# Autodesk Inventor assembly: основа
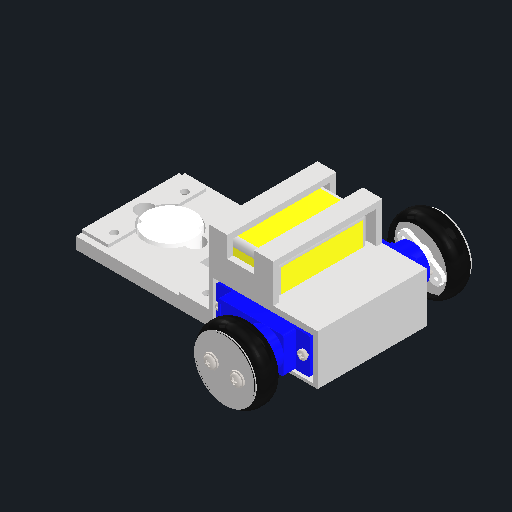
[picture p0: Inventor's stored thumbnail of the model, 512x512]
Saved by Autodesk Inventor 2022 (Build 260153000, 153)
## iProperties
Created: 2025-02-02
Part Number: основа
Document SubType Name: Assembly
Designer: Admin
Author: Admin
## Documents named in this file (7)
- D:\машина\основа.iam
- D:\abuyz lkz vfibyrb\аккум.ipt
- D:\машина\сервоприводы.iam
- D:\abuyz lkz vfibyrb\сфер.подшип.iam
- D:\машина\дно2.ipt
- D:\abuyz lkz vfibyrb\Nut GB_T 6170 M3.ipt
- D:\машина\колеса.iam
## Components (9 placed, 6 different names)
1. аккум:1
2. сервоприводы:1 [sub-assembly]
3. сферич.подш:1 [sub-assembly]
4. дно2:1
5. Nut GB/T 6170-2000 M3:1
6. Nut GB/T 6170-2000 M3:2
7. Nut GB/T 6170-2000 M3:3
8. Nut GB/T 6170-2000 M3:4
9. колеса:1 [sub-assembly]
## Relationships (31: Mate 24, Flush 7)
- [Flush]: сервоприводы:1 ↔ дно2:1
- [Mate] (0.9 mm): сервоприводы:1 ↔ дно2:1
- [Mate] (0.75 mm): сервоприводы:1 ↔ дно2:1
- [Mate] (0.75 mm): сервоприводы:1 ↔ дно2:1
- [Mate] (0.9 mm): сервоприводы:1 ↔ дно2:1
- [Flush]: сервоприводы:1 ↔ дно2:1
- [Mate] (0.5 mm): аккум:1 ↔ дно2:1
- [Flush]: аккум:1 ↔ дно2:1
- [Mate]: аккум:1 ↔ дно2:1
- [Mate]: сервоприводы:1 ↔ колеса:1
- [Mate]: сервоприводы:1 ↔ колеса:1
- [Mate]: сервоприводы:1 ↔ колеса:1
- [Mate]: сервоприводы:1 ↔ колеса:1
- [Mate]: сервоприводы:1 ↔ колеса:1
- [Mate]: сервоприводы:1 ↔ колеса:1
- [Mate]: сервоприводы:1 ↔ колеса:1
- [Mate]: сервоприводы:1 ↔ колеса:1
- [Mate]: сервоприводы:1 ↔ колеса:1
- [Mate]: сервоприводы:1 ↔ колеса:1
- [Mate]: сервоприводы:1 ↔ колеса:1
- [Mate]: сервоприводы:1 ↔ колеса:1
- [Mate]: сервоприводы:1 ↔ колеса:1
- [Mate]: сервоприводы:1 ↔ колеса:1
- [Mate]: сферич.подш:1 ↔ дно2:1
- [Mate] (5.5235 mm): сферич.подш:1 ↔ дно2:1
- [Flush]: дно2:1 ↔ Nut GB/T 6170-2000 M3:1
- [Flush]: дно2:1 ↔ Nut GB/T 6170-2000 M3:4
- [Mate]: дно2:1 ↔ Nut GB/T 6170-2000 M3:3
- [Mate]: дно2:1 ↔ Nut GB/T 6170-2000 M3:2
- [Flush]: дно2:1 ↔ Nut GB/T 6170-2000 M3:2
- [Flush]: дно2:1 ↔ Nut GB/T 6170-2000 M3:3
